# Autodesk Inventor assembly: GY_521
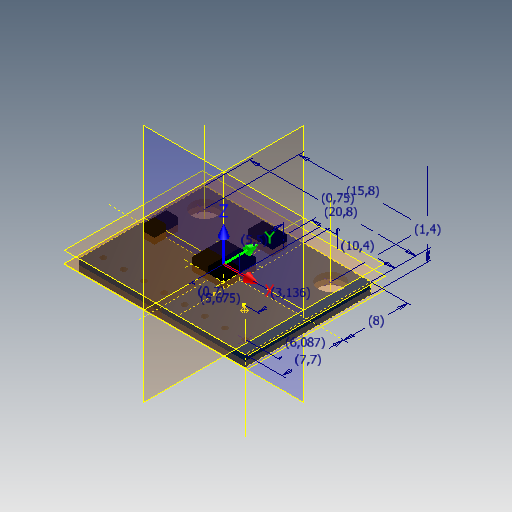
[picture p0: Inventor's stored thumbnail of the model, 512x512]
Saved by Autodesk Inventor 2021.4 (Build 254397000, 397)
## iProperties
Created: 2020-08-26
Part Number: GY_521
Material: Generisch
Document SubType Name: Assembly
Designer: ALEX
Mass: 0.469952 g
Surface Area: 8.23619 cm^2
Volume: 0.469952 cm^3
Density: 1 g/cm^3
B_Frame_Y_top: 8,000 mm
B_Frame_Y_bottom: 7,700 mm
B_Frame_X: 10,400 mm
BoardThickness: 1,400 mm
B_Frame_Z: 0,750 mm
BoardLength: 20,800 mm
Hole_Height: 5,500 mm
Fix_Hole_Width: 15,800 mm
Contact_Dist: 6,087 mm
U_BKS1_y: 3,136 mm
U_BKS1_x: 5,675 mm
U_BKS1_z: 0,700 mm
Author: ALEX
## Documents named in this file (2)
- C:\Users\alexw\Documents\Inventor\Projects\03_CurrentProjects\MasterThesis\TrainingConsol_220422\Workgroups\Workgroup_new\GY_521_v2.iam
- C:\Users\alexw\Documents\Inventor\Projects\03_CurrentProjects\MasterThesis\TrainingConsol_220422\Workgroups\Workgroup\GY_521.ipt
## Components (1 placed, 1 different names)
1. GY_521:1 — Passend:2, Fluchtend:1
## Relationships (2: Mate 1, Flush 1)
- Passend:2 [Mate]: GY_521:1
- Fluchtend:1 [Flush] (-0.75 mm): GY_521:1
## Named parameters: U_BKS1_y = 3.13554 mm, U_BKS1_x = 5.67503 mm, U_BKS1_z = 0.7 mm, B_Frame_Y_top = 8 mm, B_Frame_Y_bottom = 7.7 mm, B_Frame_X = 10.4 mm, B_Frame_Z = 0.75 mm, BoardThickness = 1.4 mm, Hole_Height = 5.5 mm, BoardLength = 20.8 mm, Fix_Hole_Width = 15.8 mm, Contact_Dist = 6.08677 mm
